# Autodesk Inventor assembly: Motor Mount Config 2
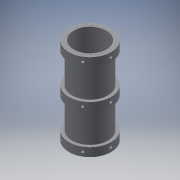
[picture p0: Inventor's stored thumbnail of the model, 180x180]
Saved by Autodesk Inventor 2019 (Build 230136000, 136)
## iProperties
Created: 2023-01-23
Part Number: Motor Mount Config 2
Document SubType Name: Assembly
Designer: user
Author: user
## Documents named in this file (3)
- C:\Users\user\Desktop\NAKUJA\Inventor Drawings\Motor Mount Config 2.iam
- C:\Users\user\Documents\Water Desalinator\Motor mount tube.ipt
- C:\Users\user\Desktop\NAKUJA\Inventor Drawings\Centering Ring.ipt
## Components (4 placed, 2 different names)
1. Centering Ring:1 — Cylindrical:3, Mate:3
2. Centering Ring:2 — Cylindrical:2, Mate:2
3. Centering Ring:3 — Cylindrical:1, Mate:1
4. Motor mount tube:1 — Cylindrical:1, Cylindrical:2, Cylindrical:3, Mate:1, Mate:2, Mate:3
## Relationships (6: CylindricalJoint 3, Mate 3)
- Cylindrical:1: Centering Ring:3 ↔ Motor mount tube:1
- Cylindrical:2: Centering Ring:2 ↔ Motor mount tube:1
- Cylindrical:3: Centering Ring:1 ↔ Motor mount tube:1
- Mate:1: Centering Ring:3 ↔ Motor mount tube:1
- Mate:2: Centering Ring:2 ↔ Motor mount tube:1
- Mate:3: Centering Ring:1 ↔ Motor mount tube:1
